# Autodesk Inventor assembly: LW bike
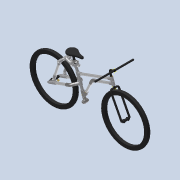
[picture p0: Inventor's stored thumbnail of the model, 180x180]
Saved by Autodesk Inventor 2021 (Build 250183000, 183)
## iProperties
RuleStatus: InUse
Created: 2020-04-29
Part Number: LW bike
Document SubType Name: Assembly
Designer: Hannah
Mass: 8355.42 g
Surface Area: 11398.8 cm^2
Volume: 1950.38 cm^3
Density: 4.28399 g/cm^3
Author: Hannah
## Documents named in this file (29)
- \\Mac\Home\Documents\GitHub\AdjustaBike-2.0\CAD\LW bike.iam
- \\Mac\Home\Documents\GitHub\AdjustaBike-2.0\CAD\prelim bike geo.ipt
- \\Mac\Home\Documents\GitHub\AdjustaBike-2.0\CAD\bottom bracket.ipt
- \\Mac\Home\Documents\GitHub\AdjustaBike-2.0\CAD\tube-09.ipt
- \\Mac\Home\Documents\GitHub\AdjustaBike-2.0\CAD\tube-11.ipt
- \\Mac\Home\Documents\GitHub\AdjustaBike-2.0\CAD\LF50-6.ipt
- \\Mac\Home\Documents\GitHub\AdjustaBike-2.0\CAD\L10-6.ipt
- \\Mac\Home\Documents\GitHub\AdjustaBike-2.0\CAD\tube-14.ipt
- \\Mac\Home\Documents\GitHub\AdjustaBike-2.0\CAD\L114-6.ipt
- \\Mac\Home\Documents\GitHub\AdjustaBike-2.0\CAD\saddle.ipt
- \\Mac\Home\Documents\GitHub\AdjustaBike-2.0\CAD\M51-5.ipt
- \\Mac\Home\Documents\GitHub\AdjustaBike-2.0\CAD\link.ipt
- \\Mac\Home\Documents\GitHub\AdjustaBike-2.0\CAD\tube-19.ipt
- \\Mac\Home\Documents\GitHub\AdjustaBike-2.0\CAD\LW head tube.ipt
- \\Mac\Home\Documents\GitHub\AdjustaBike-2.0\CAD\tube-20.ipt
- \\Mac\Home\Documents\GitHub\AdjustaBike-2.0\CAD\tube-21.ipt
- \\Mac\Home\Documents\GitHub\AdjustaBike-2.0\CAD\tube-22.ipt
- \\Mac\Home\Documents\GitHub\AdjustaBike-2.0\CAD\10-76.ipt
- \\Mac\Home\Documents\GitHub\AdjustaBike-2.0\CAD\tube-23.ipt
- \\Mac\Home\Documents\GitHub\AdjustaBike-2.0\CAD\LM50-6.ipt
- \\Mac\Home\Documents\GitHub\AdjustaBike-2.0\CAD\LM51-6.ipt
- \\Mac\Home\Documents\GitHub\AdjustaBike-2.0\CAD\55-6.ipt
- \\Mac\Home\Documents\GitHub\AdjustaBike-2.0\CAD\L21-6.ipt
- \\Mac\Home\Documents\GitHub\AdjustaBike-2.0\CAD\29-6.ipt
- \\Mac\Home\Documents\GitHub\AdjustaBike-2.0\CAD\LW sketch.ipt
- \\Mac\Home\Documents\GitHub\AdjustaBike-2.0\CAD\fasteners\DIN 1587 - M10 x 1.5.ipt
- \\Mac\Home\Documents\GitHub\AdjustaBike-2.0\CAD\fasteners\BS EN ISO 4762 - M10 x 35.ipt
- \\Mac\Home\Documents\GitHub\AdjustaBike-2.0\CAD\fasteners\BS EN ISO 4762 - M10 x 45.ipt
- \\Mac\Home\Documents\GitHub\AdjustaBike-2.0\CAD\fasteners\DIN EN ISO 7089 -  10.ipt
## Components (71 placed, 28 different names)
1. prelim bike geo:1 — Mate:1, Mate:2, Angle:1, Mate:41
2. LW sketch:1 — Mate:157, Mate:158, Mate:159, Mate:160, Mate:161, Mate:162, Mate:163, Mate:164, Mate:165, Mate:166, Mate:167, Mate:168, Mate:169, Mate:170, Mate:171, Mate:173, Mate:174, Mate:175, Mate:176, Mate:177, Mate:178, Mate:179, Flush:117, Flush:118
3. DIN 1587 - M10 x 1.5:1
4. BS EN ISO 4762 - M10 x 35:1 — Mate:220
5. DIN EN ISO 7089 -  10:1 — Mate:222
6. DIN EN ISO 7089 -  10:2 — Mate:221
7. DIN 1587 - M10 x 1.5:2
8. BS EN ISO 4762 - M10 x 35:2 — Mate:223
9. DIN EN ISO 7089 -  10:3 — Mate:224
10. DIN EN ISO 7089 -  10:4 — Mate:225
11. DIN 1587 - M10 x 1.5:4
12. BS EN ISO 4762 - M10 x 35:4 — Mate:228
13. DIN EN ISO 7089 -  10:7 — Mate:237
14. DIN EN ISO 7089 -  10:8 — Mate:229
15. DIN 1587 - M10 x 1.5:3
16. BS EN ISO 4762 - M10 x 35:3 — Mate:226
17. DIN EN ISO 7089 -  10:5 — Mate:238
18. DIN EN ISO 7089 -  10:6 — Mate:227
19. DIN 1587 - M10 x 1.5:5
20. BS EN ISO 4762 - M10 x 45:1 — Mate:233
21. DIN EN ISO 7089 -  10:9
22. DIN EN ISO 7089 -  10:10 — Mate:234
23. DIN EN ISO 7089 -  10:11
24. DIN EN ISO 7089 -  10:12
25. DIN EN ISO 7089 -  10:13 — Mate:236
26. DIN EN ISO 7089 -  10:14
27. DIN EN ISO 7089 -  10:15
28. DIN EN ISO 7089 -  10:16 — Mate:235
29. DIN 1587 - M10 x 1.5:6
30. DIN EN ISO 7089 -  10:17 — Mate:232
31. BS EN ISO 4762 - M10 x 45:2 — Mate:230
32. DIN EN ISO 7089 -  10:18 — Mate:231
33. L114-6:1 — Mate:98, Mate:99, Mate:100, Mate:163
34. LF50-6:4 — Mate:93, Mate:95, Mate:96, Mate:97, Mate:221, Mate:222
35. L10-6:3 — Mate:91, Mate:92
36. LM51-6:1 — Mate:28, Flush:16, Mate:69, Flush:20, Flush:21, Flush:22, Mate:107, Mate:110, Mate:111, Mate:112, Mate:113, Mate:114, Mate:156, Mate:228
37. L10-6:4 — Mate:15, Flush:13, Flush:14, Mate:16, Mate:179
38. L10-6:5 — Mate:17, Mate:18, Mate:156
39. L10-6:6 — Mate:13, Mate:14, Flush:11, Mate:153, Mate:178
40. L10-6:1 — Mate:82, Mate:89
41. LF50-6:2 — Mate:45, Mate:47, Angle:11, Mate:83, Flush:85, Mate:224, Mate:225
42. L21-6:1 — Mate:52, Mate:53, Mate:54, Mate:55, Mate:60
43. LF50-6:3 — Mate:69, Flush:20, Mate:98, Mate:99, Mate:108, Mate:109, Mate:162, Mate:174, Mate:230
44. LF50-6:5 — Mate:76, Mate:79, Mate:85, Mate:94, Mate:170, Flush:117, Mate:240
45. LF50-6:6 — Mate:77, Mate:78, Mate:85, Mate:86, Mate:239, Flush:118
46. LM50-6:1 — Mate:75, Mate:83, Flush:85, Mate:86, Mate:223
47. LM50-6:2 — Mate:74, Mate:94, Mate:95, Mate:96, Mate:220
48. seat tube:1 — Mate:7, Tangent:1, Flush:9, Angle:2, Mate:8, Angle:5, Mate:17, Tangent:7, Tangent:8, Mate:28, Mate:52, Flush:21, Mate:106, Tangent:11, Mate:157
49. down tube A:1 — Mate:153, Tangent:10, Mate:155, Mate:160
50. down tube B:1 — Flush:10, Angle:3, Tangent:2, Mate:152, Mate:154, Mate:159
51. top tube:1 — Mate:16, Tangent:4, Mate:18, Tangent:11, Mate:158, Mate:245
52. seatstay:1 — Mate:91, Mate:93, Mate:97, Mate:164
53. seatstay:2 — Mate:45, Mate:47, Mate:82, Tangent:9, Mate:165
54. seatstay spacer:1 — Mate:89, Mate:90, Mate:92, Mate:100, Tangent:9, Mate:175, Mate:176
55. chainstay:1 — Mate:58, Mate:62, Angle:12, Mate:75, Mate:77, Mate:166, Mate:239
56. chainstay:2 — Mate:59, Mate:64, Angle:13, Mate:74, Mate:76, Mate:167
57. chainstay spacer:1 — Tangent:8, Mate:55, Mate:57, Mate:61, Mate:169
58. chainstay spacer:2 — Tangent:7, Mate:54, Mate:56, Mate:63, Mate:168
59. LW head tube:1 — Mate:14, Flush:11, Flush:12, Angle:5, Mate:15, Flush:13, Tangent:4, Tangent:10, Mate:161, Mate:241, Mate:242
60. bottom bracket:1 — Mate:4, Flush:1, Mate:5, Mate:6, Tangent:1, Mate:171, Mate:173, Mate:177
61. saddle:1 — Mate:106, Flush:116
62. link:1 — Mate:107, Mate:109, Mate:231, Mate:234, Mate:235
63. link:2 — Mate:111, Mate:113, Mate:227, Mate:229
64. link:3 — Mate:108, Mate:112, Mate:232, Mate:236
65. link:4 — Mate:110, Mate:114, Mate:237, Mate:238
66. M51-5:1 — Mate:226, Mate:233
67. 10-76:1 — Mate:6, Flush:2, Mate:7, Mate:9
68. 29-6:1 — Mate:8, Mate:9, Mate:10, Angle:3, Tangent:2, Mate:53, Mate:150, Mate:151
69. 55-6:3 — Mate:154, Mate:155
70. 55-6:1 — Mate:56, Mate:59, Mate:63, Mate:64
71. 55-6:2 — Mate:57, Mate:58, Mate:61, Mate:62
## Relationships (197: Mate 165, Flush 17, Tangent 8, Angle 7)
- Mate:1: prelim bike geo:1
- Mate:2: prelim bike geo:1
- Mate:3
- Mate:4: bottom bracket:1
- Flush:1: bottom bracket:1
- Angle:1 (0 deg): prelim bike geo:1
- Mate:5: bottom bracket:1
- Mate:6: bottom bracket:1 ↔ 10-76:1
- Flush:2: 10-76:1
- Mate:7: seat tube:1 ↔ 10-76:1
- Tangent:1: seat tube:1 ↔ bottom bracket:1
- Flush:9: seat tube:1
- Angle:2 (-70 deg): seat tube:1
- Flush:10: down tube B:1
- Mate:8: seat tube:1 ↔ 29-6:1
- Mate:9 (5 mm): 10-76:1 ↔ 29-6:1
- Mate:10: 29-6:1
- Angle:3 (45 deg): down tube B:1 ↔ 29-6:1
- Tangent:2: down tube B:1 ↔ 29-6:1
- Mate:13: L10-6:6
- Mate:14: L10-6:6 ↔ LW head tube:1
- Flush:11: L10-6:6 ↔ LW head tube:1
- Flush:12: LW head tube:1
- Angle:5 (0 deg): seat tube:1 ↔ LW head tube:1
- Mate:15: L10-6:4 ↔ LW head tube:1
- Flush:13: L10-6:4 ↔ LW head tube:1
- Flush:14: L10-6:4
- Mate:16: L10-6:4 ↔ top tube:1
- Tangent:4: top tube:1 ↔ LW head tube:1
- Mate:17: L10-6:5 ↔ seat tube:1
- Mate:18: L10-6:5 ↔ top tube:1
- Tangent:7: seat tube:1 ↔ chainstay spacer:2
- Tangent:8: seat tube:1 ↔ chainstay spacer:1
- Mate:28: LM51-6:1 ↔ seat tube:1
- Flush:16: LM51-6:1
- Mate:41: prelim bike geo:1
- Mate:45: LF50-6:2 ↔ seatstay:2
- Mate:47: LF50-6:2 ↔ seatstay:2
- Angle:11 (0 deg): LF50-6:2
- Mate:52: L21-6:1 ↔ seat tube:1
- Mate:53 (5 mm): L21-6:1 ↔ 29-6:1
- Mate:54: L21-6:1 ↔ chainstay spacer:2
- Mate:55: L21-6:1 ↔ chainstay spacer:1
- Mate:56: chainstay spacer:2 ↔ 55-6:1
- Mate:57: chainstay spacer:1 ↔ 55-6:2
- Mate:58: chainstay:1 ↔ 55-6:2
- Mate:59: chainstay:2 ↔ 55-6:1
- Mate:60: L21-6:1
- Mate:61 (-35 mm): chainstay spacer:1 ↔ 55-6:2
- Mate:62 (-35 mm): chainstay:1 ↔ 55-6:2
- Mate:63 (-35 mm): chainstay spacer:2 ↔ 55-6:1
- Mate:64 (-35 mm): chainstay:2 ↔ 55-6:1
- Angle:12 (0 deg): chainstay:1
- Angle:13 (0 deg): chainstay:2
- Mate:69: LM51-6:1 ↔ LF50-6:3
- Flush:20: LM51-6:1 ↔ LF50-6:3
- Flush:21: LM51-6:1 ↔ seat tube:1
- Mate:74: LM50-6:2 ↔ chainstay:2
- Mate:75: LM50-6:1 ↔ chainstay:1
- Mate:76: LF50-6:5 ↔ chainstay:2
- Mate:77: LF50-6:6 ↔ chainstay:1
- Mate:78: LF50-6:6
- Mate:79: LF50-6:5
- Flush:22: LM51-6:1
- Mate:82: L10-6:1 ↔ seatstay:2
- Mate:83: LF50-6:2 ↔ LM50-6:1
- Flush:85: LF50-6:2 ↔ LM50-6:1
- Mate:85: LF50-6:5 ↔ LF50-6:6
- Mate:86 (5 mm): LF50-6:6 ↔ LM50-6:1
- Mate:89: L10-6:1 ↔ seatstay spacer:1
- Mate:90: seatstay spacer:1
- Mate:91: L10-6:3 ↔ seatstay:1
- Mate:92: L10-6:3 ↔ seatstay spacer:1
- Mate:93: LF50-6:4 ↔ seatstay:1
- Mate:94 (5 mm): LF50-6:5 ↔ LM50-6:2
- Mate:95: LF50-6:4 ↔ LM50-6:2
- Mate:96: LF50-6:4 ↔ LM50-6:2
- Mate:97: LF50-6:4 ↔ seatstay:1
- Mate:98: L114-6:1 ↔ LF50-6:3
- Mate:99: L114-6:1 ↔ LF50-6:3
- Mate:100: L114-6:1 ↔ seatstay spacer:1
- Tangent:9: seatstay:2 ↔ seatstay spacer:1
- [Mate]: saddle:1 ↔ M51-5:1
- [Mate]: link:3 ↔ M51-5:1
- [Mate]: link:4 ↔ M51-5:1
- [Mate]: link:2 ↔ M51-5:1
- [Mate]: link:1 ↔ M51-5:1
- Mate:106: seat tube:1 ↔ saddle:1
- Mate:107: LM51-6:1 ↔ link:1
- Mate:108: LF50-6:3 ↔ link:3
- Mate:109: LF50-6:3 ↔ link:1
- Mate:110: LM51-6:1 ↔ link:4
- Mate:111: LM51-6:1 ↔ link:2
- Mate:112: LM51-6:1 ↔ link:3
- Mate:113: LM51-6:1 ↔ link:2
- Mate:114: LM51-6:1 ↔ link:4
- Flush:116: saddle:1
- Mate:150: 29-6:1
- Mate:151: 29-6:1
- Mate:152: down tube B:1
- Mate:153: L10-6:6 ↔ down tube A:1
- Tangent:10: down tube A:1 ↔ LW head tube:1
- Mate:154: down tube B:1 ↔ 55-6:3
- Mate:155: down tube A:1 ↔ 55-6:3
- Mate:156 (5 mm): LM51-6:1 ↔ L10-6:5
- Tangent:11: seat tube:1 ↔ top tube:1
- Mate:157: LW sketch:1 ↔ seat tube:1
- Mate:158: LW sketch:1 ↔ top tube:1
- Mate:159: LW sketch:1 ↔ down tube B:1
- Mate:160: LW sketch:1 ↔ down tube A:1
- Mate:161: LW sketch:1 ↔ LW head tube:1
- Mate:162: LW sketch:1 ↔ LF50-6:3
- Mate:163: LW sketch:1 ↔ L114-6:1
- Mate:164: LW sketch:1 ↔ seatstay:1
- Mate:165: LW sketch:1 ↔ seatstay:2
- Mate:166: LW sketch:1 ↔ chainstay:1
- Mate:167: LW sketch:1 ↔ chainstay:2
- Mate:168: LW sketch:1 ↔ chainstay spacer:2
- Mate:169: LW sketch:1 ↔ chainstay spacer:1
- Mate:170: LW sketch:1 ↔ LF50-6:5
- Mate:171: LW sketch:1 ↔ bottom bracket:1
- Mate:173: LW sketch:1 ↔ bottom bracket:1
- Mate:174: LW sketch:1 ↔ LF50-6:3
- Mate:175: LW sketch:1 ↔ seatstay spacer:1
- Mate:176: LW sketch:1 ↔ seatstay spacer:1
- Mate:177: LW sketch:1 ↔ bottom bracket:1
- Mate:178: LW sketch:1 ↔ L10-6:6
- Mate:179: LW sketch:1 ↔ L10-6:4
- [Mate]: BS EN ISO 4762 - M10 x 35:1 ↔ DIN EN ISO 7089 -  10:1
- [Mate]: BS EN ISO 4762 - M10 x 35:1 ↔ DIN EN ISO 7089 -  10:1
- [Mate]: BS EN ISO 4762 - M10 x 35:1 ↔ DIN EN ISO 7089 -  10:2
- [Mate]: DIN 1587 - M10 x 1.5:1 ↔ BS EN ISO 4762 - M10 x 35:1
- [Mate]: DIN 1587 - M10 x 1.5:2 ↔ BS EN ISO 4762 - M10 x 35:2
- [Mate]: BS EN ISO 4762 - M10 x 35:2 ↔ DIN EN ISO 7089 -  10:3
- [Mate]: BS EN ISO 4762 - M10 x 35:2 ↔ DIN EN ISO 7089 -  10:3
- [Mate]: BS EN ISO 4762 - M10 x 35:2 ↔ DIN EN ISO 7089 -  10:4
- [Mate]: DIN 1587 - M10 x 1.5:3 ↔ BS EN ISO 4762 - M10 x 35:3
- [Mate]: BS EN ISO 4762 - M10 x 35:3 ↔ DIN EN ISO 7089 -  10:5
- [Mate]: BS EN ISO 4762 - M10 x 35:3 ↔ DIN EN ISO 7089 -  10:5
- [Mate]: BS EN ISO 4762 - M10 x 35:3 ↔ DIN EN ISO 7089 -  10:6
- [Mate]: DIN 1587 - M10 x 1.5:1 ↔ DIN EN ISO 7089 -  10:2
- [Mate]: DIN 1587 - M10 x 1.5:2 ↔ DIN EN ISO 7089 -  10:4
- [Mate]: DIN 1587 - M10 x 1.5:3 ↔ DIN EN ISO 7089 -  10:6
- [Mate]: BS EN ISO 4762 - M10 x 35:4 ↔ DIN EN ISO 7089 -  10:7
- [Mate]: BS EN ISO 4762 - M10 x 35:4 ↔ DIN EN ISO 7089 -  10:7
- [Mate]: DIN 1587 - M10 x 1.5:4 ↔ BS EN ISO 4762 - M10 x 35:4
- [Mate]: DIN 1587 - M10 x 1.5:4 ↔ DIN EN ISO 7089 -  10:8
- [Mate]: BS EN ISO 4762 - M10 x 35:4 ↔ DIN EN ISO 7089 -  10:8
- [Mate]: DIN 1587 - M10 x 1.5:5 ↔ BS EN ISO 4762 - M10 x 45:1
- [Mate]: BS EN ISO 4762 - M10 x 45:1 ↔ DIN EN ISO 7089 -  10:9
- [Mate]: BS EN ISO 4762 - M10 x 45:1 ↔ DIN EN ISO 7089 -  10:9
- [Mate]: BS EN ISO 4762 - M10 x 45:1 ↔ DIN EN ISO 7089 -  10:10
- [Mate]: DIN 1587 - M10 x 1.5:5 ↔ DIN EN ISO 7089 -  10:10
- [Mate]: BS EN ISO 4762 - M10 x 45:1 ↔ DIN EN ISO 7089 -  10:12
- [Mate]: BS EN ISO 4762 - M10 x 45:1 ↔ DIN EN ISO 7089 -  10:11
- [Mate]: BS EN ISO 4762 - M10 x 45:1 ↔ DIN EN ISO 7089 -  10:13
- [Mate]: DIN EN ISO 7089 -  10:12 ↔ DIN EN ISO 7089 -  10:13
- [Mate]: DIN EN ISO 7089 -  10:11 ↔ DIN EN ISO 7089 -  10:12
- [Mate]: DIN EN ISO 7089 -  10:14 ↔ DIN EN ISO 7089 -  10:15
- [Mate]: DIN EN ISO 7089 -  10:15 ↔ DIN EN ISO 7089 -  10:16
- [Mate]: BS EN ISO 4762 - M10 x 45:1 ↔ DIN EN ISO 7089 -  10:16
- [Mate]: BS EN ISO 4762 - M10 x 45:1 ↔ DIN EN ISO 7089 -  10:15
- [Mate]: BS EN ISO 4762 - M10 x 45:1 ↔ DIN EN ISO 7089 -  10:14
- [Mate]: DIN 1587 - M10 x 1.5:6 ↔ BS EN ISO 4762 - M10 x 45:2
- [Mate]: DIN EN ISO 7089 -  10:17 ↔ BS EN ISO 4762 - M10 x 45:2
- [Mate]: DIN EN ISO 7089 -  10:17 ↔ BS EN ISO 4762 - M10 x 45:2
- [Mate]: DIN 1587 - M10 x 1.5:6 ↔ DIN EN ISO 7089 -  10:18
- [Mate]: BS EN ISO 4762 - M10 x 45:2 ↔ DIN EN ISO 7089 -  10:18
- Mate:220: BS EN ISO 4762 - M10 x 35:1 ↔ LM50-6:2
- Mate:221: DIN EN ISO 7089 -  10:2 ↔ LF50-6:4
- Mate:222: DIN EN ISO 7089 -  10:1 ↔ LF50-6:4
- Mate:223: BS EN ISO 4762 - M10 x 35:2 ↔ LM50-6:1
- Mate:224: DIN EN ISO 7089 -  10:3 ↔ LF50-6:2
- Mate:225: DIN EN ISO 7089 -  10:4 ↔ LF50-6:2
- Mate:226: BS EN ISO 4762 - M10 x 35:3 ↔ M51-5:1
- Mate:227: DIN EN ISO 7089 -  10:6 ↔ link:2
- Mate:228: BS EN ISO 4762 - M10 x 35:4 ↔ LM51-6:1
- Mate:229: DIN EN ISO 7089 -  10:8 ↔ link:2
- Mate:230: BS EN ISO 4762 - M10 x 45:2 ↔ LF50-6:3
- Mate:231: DIN EN ISO 7089 -  10:18 ↔ link:1
- Mate:232: DIN EN ISO 7089 -  10:17 ↔ link:3
- Mate:233: BS EN ISO 4762 - M10 x 45:1 ↔ M51-5:1
- Mate:234: DIN EN ISO 7089 -  10:10 ↔ link:1
- Mate:235: DIN EN ISO 7089 -  10:16 ↔ link:1
- Mate:236: DIN EN ISO 7089 -  10:13 ↔ link:3
- Mate:237: DIN EN ISO 7089 -  10:7 ↔ link:4
- Mate:238: DIN EN ISO 7089 -  10:5 ↔ link:4
- Mate:239: LF50-6:6 ↔ chainstay:1
- Flush:117: LW sketch:1 ↔ LF50-6:5
- Flush:118: LW sketch:1 ↔ LF50-6:6
- Flush:119 (60 mm)
- Mate:240: LF50-6:5
- Mate:241: LW head tube:1
- Mate:242: LW head tube:1
- Mate:243 (538 mm)
- Mate:244 (406 mm)
- Mate:245: top tube:1
## Named parameters: Lst = 440 mm, Sst = 6, Ldt = 230 mm, Sdt = 6, Ltt = 532 mm, Stt = 6, Scs = 6, Lss = 260 mm, Sss = 6, Lsp = 78 mm, Ssp = 6, Lcs = 300 mm, Lspn = 228 mm, d166_d164 = 0 mm, Ldtb = 304 mm, d278_d304 = 0 mm, d279_d305 = 0 mm, d280_d306 = 0 mm, d281_d307 = 0 mm, d282_d308 = 0 mm, d283_d312 = 0 mm, d284_d313 = 0 mm, d285_d314 = 0 mm, d286_d316 = 0 mm, d287_d317 = 0 mm, d298_d259 = 0 mm, d299_d261 = 0 mm, d300_d262 = 0 mm, d301_d263 = 0 mm, d302_d264 = 0 mm, d303_d275 = 0 mm, d304_d276 = 0 mm, d305_d277 = 0 mm, d315_d248 = 0 mm, d316_d249 = 0 mm, d317_d254 = 0 mm, TTLength = 532.47204 mm, DTbLength = 304.32287 mm, DTaLength = 230.72851 mm, wheelbase = 1116.62191 mm, CSLength = 300 mm, stack = 538 mm, reach = 406 mm, BBdrop = 60 mm, hub_spacing = 144.28534 mm
